# Autodesk Inventor assembly: FrisbeeShooterV02
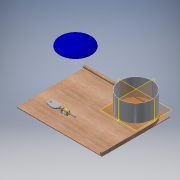
[picture p0: Inventor's stored thumbnail of the model, 180x180]
Saved by Autodesk Inventor 2019.4 (Build 234330000, 330)
## iProperties
Created: 2019-04-25
Part Number: FrisbeeShooterV02
Document SubType Name: Assembly
Designer: steele
Author: steele
## Documents named in this file (7)
- C:\git\CAD-Development\robSteele\2013FrcUltimateAscent\FrisbeeShooterV02.iam
- C:\git\CAD-Development\robSteele\2013FrcUltimateAscent\ShooterBaseV02.ipt
- C:\git\CAD-Development\robSteele\2013FrcUltimateAscent\53214-b_2013.ipt
- C:\git\CAD-Development\robSteele\2013FrcUltimateAscent\FrisbeeHopperV02.ipt
- C:\git\CAD-Development\robSteele\2013FrcUltimateAscent\FrisbeeShooterV02\Design Accelerator\Disc Cam1.iam
- C:\git\CAD-Development\robSteele\2013FrcUltimateAscent\camPostHolderV02.ipt
- C:\git\CAD-Development\robSteele\2013FrcUltimateAscent\camPostV02.ipt
## Components (6 placed, 6 different names)
1. ShooterBaseV02:1 — Insert:1, Mate:3, Flush:1, Flush:2, Mate:5, Mate:6
2. 53214-b_2013:1
3. FrisbeeHopperV02:1 — Insert:1
4. Disc Cam:1 [sub-assembly] — Tangent:1, Mate:5, Mate:6
5. camPostHolderV02:1 — Mate:3, Flush:1, Flush:2, Mate:4
6. camPostV02:1 — Mate:4, Tangent:1
## Relationships (8: Mate 4, Flush 2, Insert 1, Tangent 1)
- Insert:1 (50.8 mm): ShooterBaseV02:1 ↔ FrisbeeHopperV02:1
- Mate:3 (12.7 mm): ShooterBaseV02:1 ↔ camPostHolderV02:1
- Flush:1 (254 mm): ShooterBaseV02:1 ↔ camPostHolderV02:1
- Flush:2 (152.4 mm): ShooterBaseV02:1 ↔ camPostHolderV02:1
- Mate:4: camPostHolderV02:1 ↔ camPostV02:1
- Tangent:1: Disc Cam:1 ↔ camPostV02:1
- Mate:5: ShooterBaseV02:1 ↔ Disc Cam:1
- Mate:6 (26.9875 mm): ShooterBaseV02:1 ↔ Disc Cam:1
